# Autodesk Inventor assembly: StoragePoint_testasm
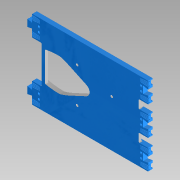
[picture p0: Inventor's stored thumbnail of the model, 180x180]
Saved by Autodesk Inventor 2021 (Build 250183000, 183)
## iProperties
Created: 2021-03-05
Part Number: StoragePoint_testasm
Document SubType Name: Assembly
Designer: kumagai
Author: kumagai
## Documents named in this file (5)
- X:\Develop\CAD\PlaRails\StoragePoint\PocketPoint_testasm.iam
- X:\Develop\CAD\PlaRails\StoragePoint\PocketPoint_C.ipt
- X:\Develop\CAD\PlaRails\StoragePoint\PocketPointBar1.ipt
- X:\Develop\CAD\PlaRails\StoragePoint\PocketPointBar1_MIR.ipt
- X:\Develop\CAD\PlaRails\StoragePoint\PocketPointBar2.ipt
## Components (4 placed, 4 different names)
1. PocketPoint_C:1 — 回転:1, 回転:2, 回転:3
2. PocketPointBar1:1 — 回転:2
3. PocketPointBar1_MIR:1 — 回転:1
4. PocketPointBar2:1 — 回転:3
## Relationships (3: RevoluteJoint 3)
- 回転:1 [RevoluteJoint]: PocketPoint_C:1 ↔ PocketPointBar1_MIR:1
- 回転:2 [RevoluteJoint]: PocketPoint_C:1 ↔ PocketPointBar1:1
- 回転:3 [RevoluteJoint]: PocketPoint_C:1 ↔ PocketPointBar2:1
